# Autodesk Inventor assembly: 01.00.00.00
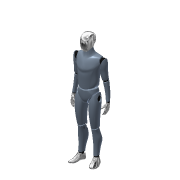
[picture p0: Inventor's stored thumbnail of the model, 180x180]
Saved by Autodesk Inventor 2016 (Build 200138000, 138)
## iProperties
Manager: GrabCad
Category: N/C
Created: 2017-03-23
Part Number: 01.00.00.00
Document SubType Name: Assembly
Designer: Wesley Perez
Project: KIT ADEBOTT - Projetos rápidos
Checked By: GrabCad
User Status: Criado item
Description: Corpo Humano em Escala
Author: Wesley Perez
Title: Corpo Humano em Escala
Subject: CAD 3D
Keywords: Altura 1.75m
Revision Number: 00
## Documents named in this file (3)
- D:\EMPRESARIAL\ADEBOTT\Dep. PROJETOS\ADEBOTT - KIT PROJETISTA\Corpos Humanos\Corpo Humano 01\01.00.00.00 - Corpo Humano.iam
- D:\EMPRESARIAL\ADEBOTT\Dep. PROJETOS\ADEBOTT - KIT PROJETISTA\Corpos Humanos\Corpo Humano 01\01.01.01.00 - Membros inferiores.iam
- D:\EMPRESARIAL\ADEBOTT\Dep. PROJETOS\ADEBOTT - KIT PROJETISTA\Corpos Humanos\Corpo Humano 01\01.02.01.00 - Membros superiores.iam
## Components (2 placed, 2 different names)
1. 01.01.01.00 - Membros inferiores:1 [sub-assembly] — Alinhamento:1, Alinhamento:2, Alinhamento:3, Coincidência:1, Alinhamento:4
2. 01.02.01.00 - Membros superiores:1 [sub-assembly] — Coincidência:1, Alinhamento:4
## Relationships (5: Flush 4, Mate 1)
- Alinhamento:1 [Flush]: 01.01.01.00 - Membros inferiores:1
- Alinhamento:2 [Flush]: 01.01.01.00 - Membros inferiores:1
- Alinhamento:3 [Flush]: 01.01.01.00 - Membros inferiores:1
- Coincidência:1 [Mate]: 01.01.01.00 - Membros inferiores:1 ↔ 01.02.01.00 - Membros superiores:1
- Alinhamento:4 [Flush]: 01.01.01.00 - Membros inferiores:1 ↔ 01.02.01.00 - Membros superiores:1
